# Autodesk Inventor assembly: Funnel Back
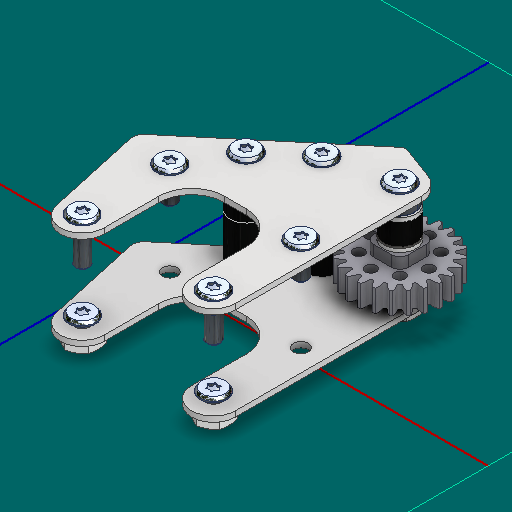
[picture p0: Inventor's stored thumbnail of the model, 512x512]
Saved by Autodesk Inventor 2025 (Build 290162000, 162)
## iProperties
Created: 2024-10-18
Part Number: Funnel Back
Document SubType Name: Assembly
Designer: averey
Author: averey
## Documents named in this file (20)
- C:\Users\avere\VEX\High Stakes\CAD\V2\Chassis\Drivebay Left\Funnel Back.iam
- C:\Users\avere\VEX\High Stakes\CAD\V2\Chassis\Drivebay Left\Custom Parts\Funnel Gusset Back.ipt
- C:\Users\avere\VEX\High Stakes\CAD\ROBOPROS-CAD-Inventor\Motion\Spacers\Spacer Nylon .375 OD\NSpacer .375 OD x .500.ipt
- C:\Users\avere\VEX\High Stakes\CAD\ROBOPROS-CAD-Inventor\Motion\Spacers\Spacer Nylon .375 OD.ipt
- C:\Users\avere\VEX\High Stakes\CAD\ROBOPROS-CAD-Inventor\Structure\Hardware\Screw Steel - Star\SScrew Star Smooth 1.250.ipt
- C:\Users\avere\VEX\High Stakes\CAD\ROBOPROS-CAD-Inventor\Structure\Hardware\Screw Steel - Star.ipt
- C:\Users\avere\VEX\High Stakes\CAD\ROBOPROS-CAD-Inventor\Structure\Hardware\Nut Nylon\Nut Nylon - White.ipt
- C:\Users\avere\VEX\High Stakes\CAD\ROBOPROS-CAD-Inventor\Structure\Hardware\Screw Shoulder Robosource\SScrew Shoulder Smooth .375 x .12.ipt
- C:\Users\avere\VEX\High Stakes\CAD\ROBOPROS-CAD-Inventor\Structure\Hardware\Screw Shoulder Robosource.ipt
- C:\Users\avere\VEX\High Stakes\CAD\ROBOPROS-CAD-Inventor\Modified Parts\Half Cut HS 24T Gear, No Insert.ipt
- C:\Users\avere\VEX\High Stakes\CAD\ROBOPROS-CAD-Inventor\Structure\Hardware\Nut Keps.ipt
- C:\Users\avere\VEX\High Stakes\CAD\ROBOPROS-CAD-Inventor\Motion\Spacers\Spacer Nylon .375 OD\NSpacer .375 OD x .250.ipt
- C:\Users\avere\VEX\High Stakes\CAD\ROBOPROS-CAD-Inventor\Motion\Spacers\Washer Teflon\TWasher .375 OD x .04000.ipt
- C:\Users\avere\VEX\High Stakes\CAD\ROBOPROS-CAD-Inventor\Motion\Spacers\Washer Steel\SWasher .375 OD x .015625.ipt
- C:\Users\avere\VEX\High Stakes\CAD\ROBOPROS-CAD-Inventor\Structure\Hardware\Screw Shoulder Robosource\SScrew Shoulder Smooth .290 x .09.ipt
- D:\VEX\High Stakes\CAD\ROBOPROS-CAD-Inventor\Structure\Hardware\Screw Shoulder Robosource.ipt
- D:\VEX\High Stakes\CAD\ROBOPROS-CAD-Inventor\Structure\Hardware\Nut Nylon.ipt
- C:\Users\avere\VEX\High Stakes\CAD\ROBOPROS-CAD-Inventor\Structure\Hardware\Screw Shoulder Robosource\SScrew Shoulder Smooth .500 x .18.ipt
- C:\Users\avere\VEX\High Stakes\CAD\ROBOPROS-CAD-Inventor\Motion\Spacers\Washer Teflon.ipt
- C:\Users\avere\VEX\High Stakes\CAD\ROBOPROS-CAD-Inventor\Motion\Spacers\Washer Steel.ipt
## Components (26 placed, 12 different names)
1. Funnel Gusset Back:1 — Mate:1, Insert:4, Insert:5, Insert:6, Insert:9, Insert:17, Insert:18, Insert:27, Insert:28
2. Funnel Gusset Back:2 — Mate:1, Insert:2, Insert:8, Insert:7, Insert:20, Insert:21, Insert:24, Insert:25, Insert:26
3. NSpacer .375 OD x .500:1 — Insert:1
4. NSpacer .375 OD x .500:2 — Insert:2, Insert:1
5. NSpacer .375 OD x .500:3 — Insert:4, Insert:3
6. NSpacer .375 OD x .500:4 — Insert:3
7. SScrew Star Smooth 1.250:1 — Insert:5
8. SScrew Star Smooth 1.250:2 — Insert:6
9. Nut Nylon - White:1 — Insert:8
10. Nut Nylon - White:2 — Insert:7
11. Half Cut HS 24T Gear, No Insert:1
12. Nut Keps:1 — Insert:18, Insert:19
13. NSpacer .375 OD x .250:5
14. TWasher .375 OD x .04000:1
15. TWasher .375 OD x .04000:2 — Insert:19
16. SWasher .375 OD x .015625:1
17. SScrew Star Smooth 1.250:3 — Insert:17
18. Nut Nylon - White:4 — Insert:20
19. SScrew Shoulder Smooth .290 x .09:8 — Insert:21
20. Nut Nylon - White:5 — Insert:24
21. Nut Nylon - White:7 — Insert:26
22. SScrew Shoulder Smooth .290 x .09:11 — Insert:25
23. SScrew Shoulder Smooth .500 x .18:12 — Insert:27
24. SScrew Shoulder Smooth .500 x .18:13 — Insert:28
25. SScrew Shoulder Smooth .375 x .12:1 — Insert:9
26. SScrew Shoulder Smooth .375 x .12:4
## Component patterns: (2 elements, first: SScrew Shoulder Smooth .375 x .12:1)
## Relationships (24: Insert 23, Mate 1)
- Mate:1: Funnel Gusset Back:1 ↔ Funnel Gusset Back:2
- Insert:2: Funnel Gusset Back:2 ↔ NSpacer .375 OD x .500:2
- Insert:1: NSpacer .375 OD x .500:1 ↔ NSpacer .375 OD x .500:2
- Insert:4: Funnel Gusset Back:1 ↔ NSpacer .375 OD x .500:3
- Insert:3: NSpacer .375 OD x .500:3 ↔ NSpacer .375 OD x .500:4
- Insert:5: Funnel Gusset Back:1 ↔ SScrew Star Smooth 1.250:1
- Insert:6: Funnel Gusset Back:1 ↔ SScrew Star Smooth 1.250:2
- Insert:8: Funnel Gusset Back:2 ↔ Nut Nylon - White:1
- Insert:7: Funnel Gusset Back:2 ↔ Nut Nylon - White:2
- Insert:9: Funnel Gusset Back:1 ↔ SScrew Shoulder Smooth .375 x .12:1
- [Insert]: NSpacer .375 OD x .250:5 ↔ TWasher .375 OD x .04000:2
- [Insert]: NSpacer .375 OD x .250:5 ↔ SWasher .375 OD x .015625:1
- [Insert]: TWasher .375 OD x .04000:1 ↔ SWasher .375 OD x .015625:1
- [Insert]: Half Cut HS 24T Gear, No Insert:1 ↔ TWasher .375 OD x .04000:1
- Insert:17: Funnel Gusset Back:1 ↔ SScrew Star Smooth 1.250:3
- Insert:18: Funnel Gusset Back:1 ↔ Nut Keps:1
- Insert:19: Nut Keps:1 ↔ TWasher .375 OD x .04000:2
- Insert:20: Funnel Gusset Back:2 ↔ Nut Nylon - White:4
- Insert:21 (1.5875 mm): Funnel Gusset Back:2 ↔ SScrew Shoulder Smooth .290 x .09:8
- Insert:24: Funnel Gusset Back:2 ↔ Nut Nylon - White:5
- Insert:25 (1.5875 mm): Funnel Gusset Back:2 ↔ SScrew Shoulder Smooth .290 x .09:11
- Insert:26: Funnel Gusset Back:2 ↔ Nut Nylon - White:7
- Insert:27: Funnel Gusset Back:1 ↔ SScrew Shoulder Smooth .500 x .18:12
- Insert:28: Funnel Gusset Back:1 ↔ SScrew Shoulder Smooth .500 x .18:13
